# Autodesk Inventor assembly: c2
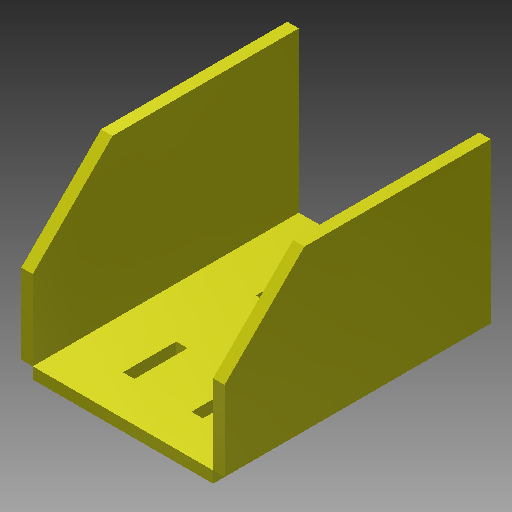
[picture p0: Inventor's stored thumbnail of the model, 512x512]
Saved by Autodesk Inventor 2017 (Build 210142000, 142)
## iProperties
Created: 2015-10-11
Part Number: c2
Document SubType Name: Assembly
Designer: daniel
Author: daniel
## Documents named in this file (3)
- C:\Users\daniel\Documents\GitHub\cardboard-stage-metric\stage\c2.iam
- C:\Users\daniel\Documents\GitHub\cardboard-stage-metric\stage\c2a.ipt
- C:\Users\daniel\Documents\GitHub\cardboard-stage-metric\stage\c2b.ipt
## Components (3 placed, 2 different names)
1. c2a:1 — Flush:1, Flush:2, Mate:1, Mate:2, Mate:3, Mate:4
2. c2b:1 — Flush:2, Mate:1, Mate:3
3. c2b:2 — Flush:1, Mate:2, Mate:4
## Relationships (6: Mate 4, Flush 2)
- Flush:1: c2a:1 ↔ c2b:2
- Flush:2: c2a:1 ↔ c2b:1
- Mate:1: c2a:1 ↔ c2b:1
- Mate:2: c2a:1 ↔ c2b:2
- Mate:3: c2a:1 ↔ c2b:1
- Mate:4: c2a:1 ↔ c2b:2
